# Autodesk Inventor assembly: wheel
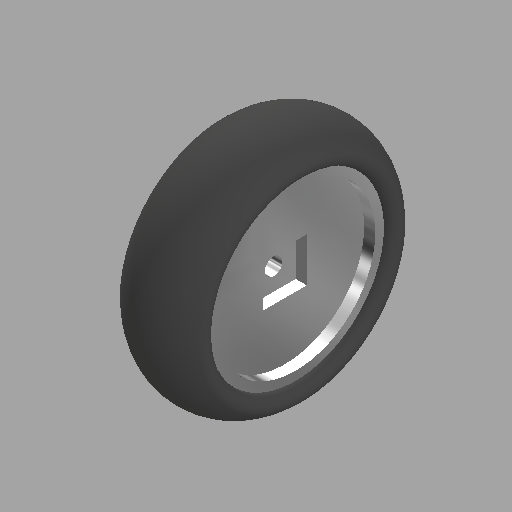
[picture p0: Inventor's stored thumbnail of the model, 512x512]
Saved by Autodesk Inventor 2024 (Build 280153000, 153)
## iProperties
Created: 2024-04-12
Part Number: wheel
Document SubType Name: Assembly
Designer: Alex
Author: Alex
## Documents named in this file (9)
- C:\Shared\alex-bartella-schoolwork\4z03\final\final\wheel.iam
- C:\Shared\alex-bartella-schoolwork\4z03\final\tire.ipt
- C:\Shared\alex-bartella-schoolwork\4z03\final\wheel.ipt
- C:\Shared\alex-bartella-schoolwork\4z03\final\final\wheel\AIP\FEA\eo2zc8a74.fins
- C:\Shared\alex-bartella-schoolwork\4z03\final\final\wheel\AIP\FEA\eo2zc8a74.fsat
- C:\Shared\alex-bartella-schoolwork\4z03\final\final\wheel\AIP\FEA\eo2zc8a74.ftes
- C:\Shared\alex-bartella-schoolwork\4z03\final\final\wheel\AIP\FEA\eo2zc8a74.fwiz
- C:\Shared\alex-bartella-schoolwork\4z03\final\final\wheel\AIP\FEA\eo2zc8a80.fmsh
- C:\Shared\alex-bartella-schoolwork\4z03\final\final\wheel\AIP\FEA\eo2zc8a81.fres
## Components (2 placed, 2 different names)
1. tire:1 — Mate:1, Mate:2, Flush:1
2. wheel:1 — Mate:1, Mate:2, Flush:1
## Relationships (3: Mate 2, Flush 1)
- Mate:1: tire:1 ↔ wheel:1
- Mate:2: tire:1 ↔ wheel:1
- Flush:1: tire:1 ↔ wheel:1
## Named parameters: sa_0 = 2200
note: some values were not read from the file. Shown as the stored number, unit unknown: "sa_0".
